# Autodesk Inventor assembly: Montagem da Câmera de Apoio ao Cilindro
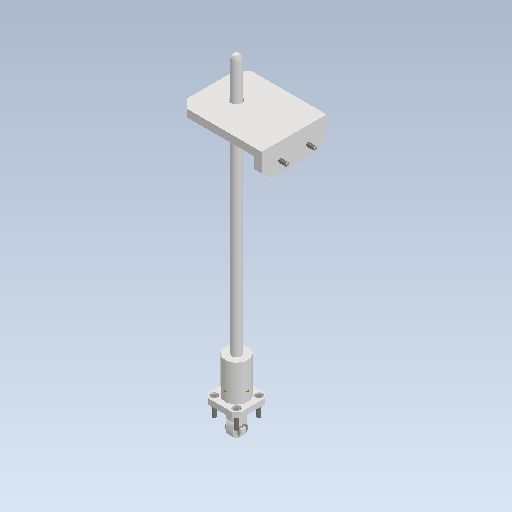
[picture p0: Inventor's stored thumbnail of the model, 512x512]
Saved by Autodesk Inventor 2021 (Build 250183000, 183)
## iProperties
Category: 10
Company: UFABC
Created: 2021-07-23
Document SubType Name: Assembly
Designer: Giovanni
Checked By: Prof. Luis
User Status: 1:4
Author: Giovanni
Title: Montagem da Câmera de Apoio ao Cilindro
Keywords: 8
## Documents named in this file (9)
- C:\Users\irineu\Documents\Inventor\MotorRadial7\Conexão2.iam
- C:\Users\irineu\Documents\Inventor\MotorRadial7\Peça28.ipt
- C:\Users\irineu\Documents\Inventor\MotorRadial7\Peça17.ipt
- C:\Users\irineu\Documents\Inventor\MotorRadial7\Peça32.ipt
- C:\Users\irineu\Documents\Inventor\MotorRadial7\Peça29.2.ipt
- C:\Users\irineu\Documents\Inventor\MotorRadial7\Peça30.ipt
- C:\Users\irineu\Documents\Inventor\MotorRadial7\Peça31.ipt
- C:\Users\irineu\Documents\Inventor\Content Center Files\R2021\pt-BR\DIN 6799\DIN 6799 - 5 6.ipt
- C:\Users\irineu\Documents\Inventor\Content Center Files\R2021\pt-BR\DIN 912\DIN 912 - M4 x 0,7 x 16 x 14,25.ipt
## Components (14 placed, 8 different names)
1. Peça28:1 — Coincidente:1, Coincidente:2, Coincidente:4, Coincidente:5, Coincidente:7, Inserir:3
2. Peça17:1 — Coincidente:1, Coincidente:2, Coincidente:3
3. Peça32:1 — Coincidente:3, Coincidente:4, Coincidente:5, Coincidente:6, Coincidente:8, Coincidente:9
4. Peça29.2:1 — Coincidente:6, Ângulo:1, Coincidente:7, Inserir:4
5. Peça30:1 — Coincidente:8, Coincidente:9, Coincidente:10, Coincidente:11, Inserir:1, Inserir:2
6. Peça31:1 — Coincidente:10, Coincidente:11
7. DIN 6799 5:1 — Inserir:1
8. DIN 6799 5:2 — Inserir:2
9. DIN 912 - substituído por DIN EN ISO 4762 M4 x 16:1 — Inserir:3
10. DIN 912 - substituído por DIN EN ISO 4762 M4 x 16:3
11. DIN 912 - substituído por DIN EN ISO 4762 M4 x 16:4
12. DIN 912 - substituído por DIN EN ISO 4762 M4 x 16:5
13. DIN 912 - substituído por DIN EN ISO 4762 M4 x 16:2 — Inserir:4
14. DIN 912 - substituído por DIN EN ISO 4762 M4 x 16:6
## Component patterns: (4 elements, first: DIN 912 - substituído por DIN EN ISO 4762 M4 x 16:1), (2 elements, first: DIN 912 - substituído por DIN EN ISO 4762 M4 x 16:2)
## Relationships (16: Mate 11, Insert 4, Angle 1)
- Coincidente:1 [Mate]: Peça28:1 ↔ Peça17:1
- Coincidente:2 [Mate]: Peça28:1 ↔ Peça17:1
- Coincidente:3 [Mate]: Peça17:1 ↔ Peça32:1
- Coincidente:4 [Mate]: Peça28:1 ↔ Peça32:1
- Coincidente:5 [Mate]: Peça28:1 ↔ Peça32:1
- Coincidente:6 [Mate]: Peça32:1 ↔ Peça29.2:1
- Ângulo:1 [Angle] (0 deg): Peça29.2:1
- Coincidente:7 [Mate] (267.5 mm): Peça28:1 ↔ Peça29.2:1
- Coincidente:8 [Mate]: Peça32:1 ↔ Peça30:1
- Coincidente:9 [Mate]: Peça32:1 ↔ Peça30:1
- Coincidente:10 [Mate]: Peça30:1 ↔ Peça31:1
- Coincidente:11 [Mate]: Peça30:1 ↔ Peça31:1
- Inserir:1: Peça30:1 ↔ DIN 6799 5:1
- Inserir:2: Peça30:1 ↔ DIN 6799 5:2
- Inserir:3: Peça28:1 ↔ DIN 912 - substituído por DIN EN ISO 4762 M4 x 16:1
- Inserir:4: Peça29.2:1 ↔ DIN 912 - substituído por DIN EN ISO 4762 M4 x 16:2
